# Autodesk Inventor assembly: Pierna
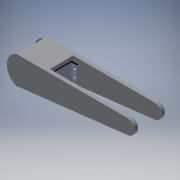
[picture p0: Inventor's stored thumbnail of the model, 180x180]
Saved by Autodesk Inventor 2018 (Build 220112000, 112)
## iProperties
Created: 2020-03-06
Part Number: Pierna
Document SubType Name: Assembly
Designer: GonzaloDiaz
Author: GonzaloDiaz
## Documents named in this file (5)
- E:\Universidad\Codigo\Enigma\Diseños\Pierna.iam
- E:\Universidad\Codigo\Enigma\Diseños\SERVOMG996R.ipt
- E:\Universidad\Codigo\Enigma\Diseños\Tibia.ipt
- E:\Universidad\Codigo\Enigma\Diseños\leva servo motore.ipt
- leva.ipt
## Components (3 placed, 3 different names)
1. SERVOMG996R:1 — Insert:1, Mate:1, Mate:2, Mate:3
2. Tibia:1 — Mate:1, Mate:2, Mate:3
3. leva:1 — Insert:1
## Relationships (4: Mate 3, Insert 1)
- Insert:1: SERVOMG996R:1 ↔ leva:1
- Mate:1: SERVOMG996R:1 ↔ Tibia:1
- Mate:2: SERVOMG996R:1 ↔ Tibia:1
- Mate:3: SERVOMG996R:1 ↔ Tibia:1
